# Autodesk Inventor assembly: WheelAssembly_v9
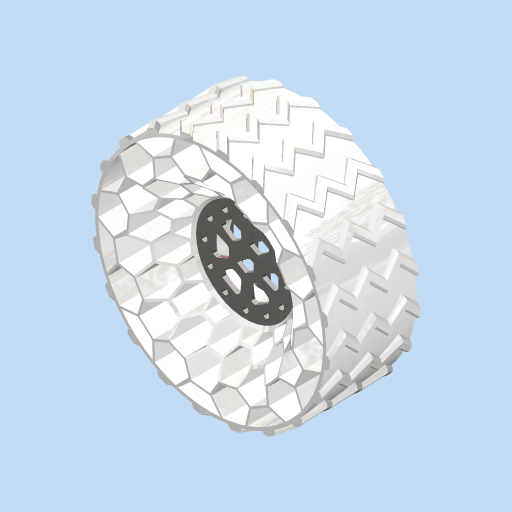
[picture p0: Inventor's stored thumbnail of the model, 512x512]
Saved by Autodesk Inventor 2023 (Build 270158000, 158)
## iProperties
Created: 2023-04-22
Part Number: WheelAssembly_v9
Document SubType Name: Assembly
Designer: asach
Author: asach
## Documents named in this file (3)
- C:\Github\BehrendURC\CAD\Chassis V3\Wheel\WheelAssembly_v9.iam
- C:\Github\BehrendURC\CAD\Chassis V3\Wheel\Tire_v9.ipt
- C:\Github\BehrendURC\CAD\Chassis V3\Wheel\ThickWheelPlate_v8.ipt
## Components (3 placed, 2 different names)
1. Tire_v9:1 — Mate:1, Mate:2, Mate:3, Mate:4, Mate:5, Mate:6
2. ThickWheelPlate_v8:1 — Mate:1, Mate:2, Mate:3
3. ThickWheelPlate_v8:2 — Mate:4, Mate:5, Mate:6
## Relationships (6: Mate 6)
- Mate:1: Tire_v9:1 ↔ ThickWheelPlate_v8:1
- Mate:2: Tire_v9:1 ↔ ThickWheelPlate_v8:1
- Mate:3: Tire_v9:1 ↔ ThickWheelPlate_v8:1
- Mate:4: Tire_v9:1 ↔ ThickWheelPlate_v8:2
- Mate:5: Tire_v9:1 ↔ ThickWheelPlate_v8:2
- Mate:6: Tire_v9:1 ↔ ThickWheelPlate_v8:2
